# Autodesk Inventor assembly: Chassis
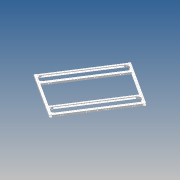
[picture p0: Inventor's stored thumbnail of the model, 180x180]
Saved by Autodesk Inventor 2014 SP1 (Build 180222100, 222)
## iProperties
Created: 2013-12-17
Part Number: Chassis
Document SubType Name: Assembly
Designer: Pradhan Alexander
Author: Pradhan Alexander
## Documents named in this file (4)
- \\STUCLUSTER\Shared\MHS\Technology\Holliday B\Group Projects\Robotics\CAD Team\CAD Team 2014\Tank Drive Chassis\Chassis.iam
- \\STUCLUSTER\Shared\MHS\Technology\Holliday B\Group Projects\Robotics\CAD Team\CAD Team 2014\Tank Drive Chassis\Chassis_Channel_AndyMark_am-0202.ipt
- \\STUCLUSTER\Shared\MHS\Technology\Holliday B\Group Projects\Robotics\CAD Team\CAD Team 2014\Tank Drive Chassis\Chassis_Channel_AndyMark_am-0202-27in.ipt
- \\STUCLUSTER\Shared\MHS\Technology\Holliday B\Group Projects\Robotics\CAD Team\CAD Team 2014\Tank Drive Chassis\Chassis_CornerConnect_AndyMark_am-0212.ipt
## Components (14 placed, 3 different names)
1. Chassis_Channel_AndyMark_am-0202:1 — Insert:9, Insert:10, Insert:11, Insert:12, Flush:19, Flush:20
2. Chassis_Channel_AndyMark_am-0202:2 — Insert:13, Insert:14, Insert:15, Insert:16, Flush:16, Flush:17, Flush:18
3. Chassis_Channel_AndyMark_am-0202:3 — Mate:2, Flush:3, Flush:4, Flush:7, Flush:8, Insert:1, Insert:2, Insert:3, Insert:4, Flush:10, Flush:14, Flush:15, Flush:18
4. Chassis_Channel_AndyMark_am-0202:4 — Mate:1, Flush:1, Flush:2, Mate:3, Flush:5, Flush:6, Flush:9, Insert:5, Insert:6, Flush:12, Flush:13
5. Chassis_Channel_AndyMark_am-0202-27in:1 — Mate:1, Flush:1, Mate:2, Flush:2, Flush:3, Flush:4, Flush:9, Flush:10, Flush:11, Insert:7, Insert:8, Insert:18, Insert:20, Flush:14, Flush:16, Flush:19
6. Chassis_Channel_AndyMark_am-0202-27in:2 — Mate:3, Flush:5, Flush:6, Flush:7, Flush:8, Flush:11, Flush:12, Flush:13, Insert:17, Insert:19, Flush:15, Flush:17, Flush:20
7. Chassis_CornerConnect_AndyMark_am-0212:1 — Insert:9, Insert:10, Insert:19
8. Chassis_CornerConnect_AndyMark_am-0212:2 — Insert:11, Insert:12, Insert:20
9. Chassis_CornerConnect_AndyMark_am-0212:3 — Insert:7, Insert:8
10. Chassis_CornerConnect_AndyMark_am-0212:4 — Insert:5, Insert:6
11. Chassis_CornerConnect_AndyMark_am-0212:5 — Insert:3, Insert:4
12. Chassis_CornerConnect_AndyMark_am-0212:6 — Insert:13, Insert:14, Insert:18
13. Chassis_CornerConnect_AndyMark_am-0212:7 — Insert:15, Insert:16, Insert:17
14. Chassis_CornerConnect_AndyMark_am-0212:8 — Insert:1, Insert:2
## Relationships (43: Flush 20, Insert 20, Mate 3)
- Mate:1: Chassis_Channel_AndyMark_am-0202:4 ↔ Chassis_Channel_AndyMark_am-0202-27in:1
- Flush:1: Chassis_Channel_AndyMark_am-0202:4 ↔ Chassis_Channel_AndyMark_am-0202-27in:1
- Mate:2: Chassis_Channel_AndyMark_am-0202:3 ↔ Chassis_Channel_AndyMark_am-0202-27in:1
- Flush:2: Chassis_Channel_AndyMark_am-0202:4 ↔ Chassis_Channel_AndyMark_am-0202-27in:1
- Flush:3: Chassis_Channel_AndyMark_am-0202:3 ↔ Chassis_Channel_AndyMark_am-0202-27in:1
- Flush:4: Chassis_Channel_AndyMark_am-0202:3 ↔ Chassis_Channel_AndyMark_am-0202-27in:1
- Mate:3: Chassis_Channel_AndyMark_am-0202:4 ↔ Chassis_Channel_AndyMark_am-0202-27in:2
- Flush:5: Chassis_Channel_AndyMark_am-0202:4 ↔ Chassis_Channel_AndyMark_am-0202-27in:2
- Flush:6: Chassis_Channel_AndyMark_am-0202:4 ↔ Chassis_Channel_AndyMark_am-0202-27in:2
- Flush:7: Chassis_Channel_AndyMark_am-0202:3 ↔ Chassis_Channel_AndyMark_am-0202-27in:2
- Flush:8: Chassis_Channel_AndyMark_am-0202:3 ↔ Chassis_Channel_AndyMark_am-0202-27in:2
- Insert:1: Chassis_Channel_AndyMark_am-0202:3 ↔ Chassis_CornerConnect_AndyMark_am-0212:8
- Insert:2: Chassis_Channel_AndyMark_am-0202:3 ↔ Chassis_CornerConnect_AndyMark_am-0212:8
- Insert:3: Chassis_Channel_AndyMark_am-0202:3 ↔ Chassis_CornerConnect_AndyMark_am-0212:5
- Insert:4: Chassis_Channel_AndyMark_am-0202:3 ↔ Chassis_CornerConnect_AndyMark_am-0212:5
- Flush:9: Chassis_Channel_AndyMark_am-0202:4 ↔ Chassis_Channel_AndyMark_am-0202-27in:1
- Flush:10: Chassis_Channel_AndyMark_am-0202:3 ↔ Chassis_Channel_AndyMark_am-0202-27in:1
- Flush:11: Chassis_Channel_AndyMark_am-0202-27in:1 ↔ Chassis_Channel_AndyMark_am-0202-27in:2
- Insert:5: Chassis_Channel_AndyMark_am-0202:4 ↔ Chassis_CornerConnect_AndyMark_am-0212:4
- Insert:6: Chassis_Channel_AndyMark_am-0202:4 ↔ Chassis_CornerConnect_AndyMark_am-0212:4
- Flush:12: Chassis_Channel_AndyMark_am-0202:4 ↔ Chassis_Channel_AndyMark_am-0202-27in:2
- Flush:13: Chassis_Channel_AndyMark_am-0202:4 ↔ Chassis_Channel_AndyMark_am-0202-27in:2
- Insert:7: Chassis_Channel_AndyMark_am-0202-27in:1 ↔ Chassis_CornerConnect_AndyMark_am-0212:3
- Insert:8: Chassis_Channel_AndyMark_am-0202-27in:1 ↔ Chassis_CornerConnect_AndyMark_am-0212:3
- Insert:9: Chassis_Channel_AndyMark_am-0202:1 ↔ Chassis_CornerConnect_AndyMark_am-0212:1
- Insert:10: Chassis_Channel_AndyMark_am-0202:1 ↔ Chassis_CornerConnect_AndyMark_am-0212:1
- Insert:11: Chassis_Channel_AndyMark_am-0202:1 ↔ Chassis_CornerConnect_AndyMark_am-0212:2
- Insert:12: Chassis_Channel_AndyMark_am-0202:1 ↔ Chassis_CornerConnect_AndyMark_am-0212:2
- Insert:13: Chassis_Channel_AndyMark_am-0202:2 ↔ Chassis_CornerConnect_AndyMark_am-0212:6
- Insert:14: Chassis_Channel_AndyMark_am-0202:2 ↔ Chassis_CornerConnect_AndyMark_am-0212:6
- Insert:15: Chassis_Channel_AndyMark_am-0202:2 ↔ Chassis_CornerConnect_AndyMark_am-0212:7
- Insert:16: Chassis_Channel_AndyMark_am-0202:2 ↔ Chassis_CornerConnect_AndyMark_am-0212:7
- Insert:17: Chassis_Channel_AndyMark_am-0202-27in:2 ↔ Chassis_CornerConnect_AndyMark_am-0212:7
- Insert:18: Chassis_Channel_AndyMark_am-0202-27in:1 ↔ Chassis_CornerConnect_AndyMark_am-0212:6
- Insert:19: Chassis_Channel_AndyMark_am-0202-27in:2 ↔ Chassis_CornerConnect_AndyMark_am-0212:1
- Insert:20: Chassis_Channel_AndyMark_am-0202-27in:1 ↔ Chassis_CornerConnect_AndyMark_am-0212:2
- Flush:14: Chassis_Channel_AndyMark_am-0202:3 ↔ Chassis_Channel_AndyMark_am-0202-27in:1
- Flush:15: Chassis_Channel_AndyMark_am-0202:3 ↔ Chassis_Channel_AndyMark_am-0202-27in:2
- Flush:16: Chassis_Channel_AndyMark_am-0202:2 ↔ Chassis_Channel_AndyMark_am-0202-27in:1
- Flush:17: Chassis_Channel_AndyMark_am-0202:2 ↔ Chassis_Channel_AndyMark_am-0202-27in:2
- Flush:18: Chassis_Channel_AndyMark_am-0202:2 ↔ Chassis_Channel_AndyMark_am-0202:3
- Flush:19: Chassis_Channel_AndyMark_am-0202:1 ↔ Chassis_Channel_AndyMark_am-0202-27in:1
- Flush:20: Chassis_Channel_AndyMark_am-0202:1 ↔ Chassis_Channel_AndyMark_am-0202-27in:2
